# Autodesk Inventor assembly: EPS
(part 2 of 2)
- Mate:673 (12.9 mm): 21-4754:3
- Mate:674 (-12.5 mm): 21-4754:4
- Mate:675 (16.2 mm): 21-4754:4
- Mate:676: 21-1002:1 ↔ EPS_PCB:1
- Mate:677: 21-1002:2 ↔ EPS_PCB:1
- Mate:678: 21-1002:3 ↔ EPS_PCB:1
- Mate:679: 21-1002:4 ↔ EPS_PCB:1
- Mate:680 (-0.3 mm): 21-1002:1
- Mate:681 (63 mm): 21-1002:1
- Mate:682 (-10 mm): 21-1002:2
- Mate:683 (21.2 mm): 21-1002:2
- Mate:684 (16.7 mm): 21-1002:3
- Flush:62 (16.4 mm): 21-1002:3
- Mate:685 (11.3 mm): 21-1002:4
- Mate:686 (89.5 mm): 21-1002:4
- Mate:687: 21-1500:1 ↔ EPS_PCB:1
- Mate:688: 21-1500:2 ↔ EPS_PCB:1
- Mate:689 (-38.6 mm): 21-1500:1
- Mate:690 (46.6 mm): 21-1500:1
- Mate:691 (44.2 mm): 21-1500:2
- Flush:63 (-30.8 mm): 21-1500:2
- Mate:692: 21-1583:1 ↔ EPS_PCB:1
- Mate:693 (-8.9 mm): 21-1583:1
- Mate:694 (84.9 mm): 21-1583:1
- Mate:695: 21-3300:1 ↔ EPS_PCB:1
- Mate:696: 21-3300:2 ↔ EPS_PCB:1
- Mate:697: 21-3603:1 ↔ EPS_PCB:1
- Mate:698: 21-3603:2 ↔ EPS_PCB:1
- Mate:699 (13.5 mm): 21-3300:1
- Flush:64 (-3.1 mm): 21-3300:1
- Mate:700 (9.5 mm): 21-3300:2
- Flush:65 (12.8 mm): 21-3300:2
- Mate:701 (54.1 mm): 21-3603:1
- Flush:66 (-35.9 mm): 21-3603:1
- Mate:702 (-29.7 mm): 21-3603:2
- Mate:703 (58.8 mm): 21-3603:2
- Mate:704: 21-4700:1 ↔ EPS_PCB:1
- Mate:705: 21-4700:2 ↔ EPS_PCB:1
- Mate:706 (37.1 mm): 21-4700:1
- Mate:707 (82.7 mm): 21-4700:1
- Mate:708 (5.2 mm): 21-4700:2
- Flush:67 (43.6 mm): 21-4700:2
- Mate:709: 21-5363:1 ↔ EPS_PCB:1
- Mate:710: 21-6203:1 ↔ EPS_PCB:1
- Mate:711: 21-6203:2 ↔ EPS_PCB:1
- Mate:712: 21-7500:1 ↔ EPS_PCB:1
- Mate:713: 21-7500:2 ↔ EPS_PCB:1
- Mate:714: 21-7500:3 ↔ EPS_PCB:1
- Mate:715: 21-7500:4 ↔ EPS_PCB:1
- Mate:716: 21-7500:5 ↔ EPS_PCB:1
- Mate:717: 21-7500:6 ↔ EPS_PCB:1
- Mate:718 (87.2 mm): 21-5363:1
- Flush:68 (-12.1 mm): 21-5363:1
- Mate:719 (54.1 mm): 21-6203:1
- Flush:69 (-39.3 mm): 21-6203:1
- Mate:720 (55.7 mm): 21-6203:2
- Flush:70 (26.9 mm): 21-6203:2
- Mate:721 (6.7 mm): 21-7500:1
- Mate:722 (21 mm): 21-7500:1
- Mate:723 (4.7 mm): 21-7500:2
- Mate:724 (28.8 mm): 21-7500:2
- Mate:725 (58.5 mm): 21-7500:3
- Flush:71 (-4.2 mm): 21-7500:3
- Mate:726 (57.1 mm): 21-7500:4
- Flush:72 (14.4 mm): 21-7500:4
- Mate:727 (26.7 mm): 21-7500:5
- Mate:728 (21 mm): 21-7500:5
- Mate:729 (21.3 mm): 21-7500:6
- Mate:730 (28.8 mm): 21-7500:6
- Mate:731: 26-0007:1 ↔ EPS_PCB:1
- Mate:732: 26-0007:2 ↔ EPS_PCB:1
- Mate:733: 26-0007:3 ↔ EPS_PCB:1
- Mate:734: 26-0007:4 ↔ EPS_PCB:1
- Mate:735: 26-0007:5 ↔ EPS_PCB:1
- Mate:736: 26-0007:6 ↔ EPS_PCB:1
- Mate:737: 26-0007:7 ↔ EPS_PCB:1
- Mate:738: 26-0007:8 ↔ EPS_PCB:1
- Mate:739: 26-0007:9 ↔ EPS_PCB:1
- Mate:740: 26-0007:10 ↔ EPS_PCB:1
- Mate:741: 26-0007:11 ↔ EPS_PCB:1
- Mate:742: 26-0007:12 ↔ EPS_PCB:1
- Mate:743: 26-0007:13 ↔ EPS_PCB:1
- Mate:744: 26-0007:14 ↔ EPS_PCB:1
- Mate:745: 26-0007:15 ↔ EPS_PCB:1
- Mate:746: 26-0007:16 ↔ EPS_PCB:1
- Mate:747 (39.2 mm): 26-0007:1
- Flush:73 (39.8 mm): 26-0007:1
- Mate:748 (-25.6 mm): 26-0007:2
- Mate:749 (79.9 mm): 26-0007:2
- Mate:750 (-10 mm): 26-0007:3
- Mate:751 (79.6 mm): 26-0007:3
- Mate:752 (28 mm): 26-0007:4
- Flush:74 (43.4 mm): 26-0007:4
- Mate:753 (23.3 mm): 26-0007:5
- Mate:754 (73 mm): 26-0007:5
- Mate:755 (23.3 mm): 26-0007:6
- Mate:756 (70.1 mm): 26-0007:6
- Mate:757 (26.1 mm): 26-0007:7
- Mate:758 (70.1 mm): 26-0007:7
- Mate:759 (26.1 mm): 26-0007:8
- Mate:760 (73 mm): 26-0007:8
- Mate:761 (20.5 mm): 26-0007:9
- Mate:762 (73 mm): 26-0007:9
- Mate:763 (33.2 mm): 26-0007:10
- Flush:75 (34.4 mm): 26-0007:10
- Mate:764 (36.2 mm): 26-0007:11
- Flush:76 (38.1 mm): 26-0007:11
- Mate:765 (30.4 mm): 26-0007:12
- Flush:77 (35.3 mm): 26-0007:12
- Mate:766 (33.2 mm): 26-0007:13
- Flush:78 (37.3 mm): 26-0007:13
- Mate:767 (-7.2 mm): 26-0007:14
- Mate:768 (79.6 mm): 26-0007:14
- Mate:769 (-12.8 mm): 26-0007:15
- Mate:770 (79.6 mm): 26-0007:15
- Mate:771 (-22.8 mm): 26-0007:16
- Mate:772 (79.9 mm): 26-0007:16
- Mate:774: 26-0000:2 ↔ EPS_PCB:1
- Mate:775: 26-0000:3 ↔ EPS_PCB:1
- Mate:776: 26-0000:1 ↔ EPS_PCB:1
- Mate:777 (-9 mm): 26-0000:1
- Flush:79 (-8 mm): 26-0000:1
- Mate:778 (-34.6 mm): 26-0000:2
- Mate:779 (76.9 mm): 26-0000:2
- Mate:780 (-9 mm): 26-0000:3
- Flush:80 (-11.1 mm): 26-0000:3
- Mate:781: 26-0001:1 ↔ EPS_PCB:1
- Mate:782: 26-0001:2 ↔ EPS_PCB:1
- Mate:783 (14.8 mm): 26-0001:1
- Flush:81 (35.2 mm): 26-0001:1
- Mate:784 (56.9 mm): 26-0001:2
- Flush:82 (-23.9 mm): 26-0001:2
- Mate:785: 26-0008:1 ↔ EPS_PCB:1
- Mate:786: 26-0008:2 ↔ EPS_PCB:1
- Mate:787: 26-0008:3 ↔ EPS_PCB:1
- Mate:788: 26-0008:4 ↔ EPS_PCB:1
- Mate:789: 26-0008:5 ↔ EPS_PCB:1
- Mate:790: 26-0008:6 ↔ EPS_PCB:1
- Mate:791: 26-0008:7 ↔ EPS_PCB:1
- Mate:792: 26-0008:8 ↔ EPS_PCB:1
- Mate:793: 26-0008:9 ↔ EPS_PCB:1
- Mate:794: 26-0008:10 ↔ EPS_PCB:1
- Mate:795: 26-0008:11 ↔ EPS_PCB:1
- Mate:796: 26-0008:12 ↔ EPS_PCB:1
- Mate:797 (8.1 mm): 26-0008:1
- Mate:798 (-43.9 mm): 26-0008:1
- Mate:799 (79.9 mm): 26-0008:2
- Mate:800 (-4.9 mm): 26-0008:2
- Mate:801 (16.6 mm): 26-0008:3
- Mate:802 (-4.8 mm): 26-0008:3
- Mate:803 (43.44 mm): 26-0008:4
- Flush:83 (-87.2 mm): 26-0008:4
- Mate:804 (88.6 mm): 26-0008:5
- Mate:805 (-44 mm): 26-0008:5
- Mate:806 (51.3 mm): 26-0008:6
- Mate:807 (27.1 mm): 26-0008:6
- Mate:808 (53.6 mm): 26-0008:7
- Mate:809 (-34.4 mm): 26-0008:7
- Mate:810 (-10.5 mm): 26-0008:8
- Flush:84 (-43.1 mm): 26-0008:8
- Mate:811 (29.4 mm): 26-0008:9
- Mate:812 (19 mm): 26-0008:9
- Mate:813 (21.3 mm): 26-0008:10
- Mate:814 (43.9 mm): 26-0008:10
- Mate:815 (62.3 mm): 26-0008:11
- Mate:816 (-32 mm): 26-0008:11
- Mate:817 (66.4 mm): 26-0008:12
- Mate:818 (40.6 mm): 26-0008:12
- Mate:819: 26-0008:13 ↔ EPS_PCB:1
- Mate:820: 26-0008:14 ↔ EPS_PCB:1
- Mate:821 (35.5 mm): 26-0008:13
- Flush:85 (14.8 mm): 26-0008:13
- Mate:822 (58.5 mm): 26-0008:14
- Flush:86 (-27.2 mm): 26-0008:14
- Mate:823: 11-105A:1 ↔ EPS_PCB:1
- Mate:824: 11-105A:2 ↔ EPS_PCB:1
- Mate:825: 11-105A:3 ↔ EPS_PCB:1
- Mate:826: 11-105A:4 ↔ EPS_PCB:1
- Mate:827: 11-105A:5 ↔ EPS_PCB:1
- Mate:828: 11-105A:6 ↔ EPS_PCB:1
- Mate:829: 11-105A:7 ↔ EPS_PCB:1
- Mate:830: 11-105A:8 ↔ EPS_PCB:1
- Mate:831: 11-105A:9 ↔ EPS_PCB:1
- Mate:832: 11-105A:10 ↔ EPS_PCB:1
- Mate:833: 11-105A:11 ↔ EPS_PCB:1
- Mate:834: 11-105A:12 ↔ EPS_PCB:1
- Mate:835: 11-105A:13 ↔ EPS_PCB:1
- Mate:836: 11-105A:14 ↔ EPS_PCB:1
- Mate:837: 11-105A:15 ↔ EPS_PCB:1
- Mate:838: 11-105A:16 ↔ EPS_PCB:1
- Mate:839: 11-105A:17 ↔ EPS_PCB:1
- Mate:840: 11-105A:18 ↔ EPS_PCB:1
- Mate:841: 11-105A:19 ↔ EPS_PCB:1
- Mate:842: 11-105A:20 ↔ EPS_PCB:1
- Mate:843: 11-105A:21 ↔ EPS_PCB:1
- Mate:844: 11-105A:22 ↔ EPS_PCB:1
- Mate:845: 11-105A:23 ↔ EPS_PCB:1
- Mate:846: 11-105A:24 ↔ EPS_PCB:1
- Mate:847: 11-105A:25 ↔ EPS_PCB:1
- Mate:848: 11-105A:26 ↔ EPS_PCB:1
- Mate:849 (37.6 mm): 11-105A:1
- Mate:850 (32.9 mm): 11-105A:1
- Mate:851 (40.9 mm): 11-105A:2
- Mate:852 (18.8 mm): 11-105A:2
- Mate:853 (-5.5 mm): 11-105A:3
- Flush:87 (-25.8 mm): 11-105A:3
- Mate:854 (-43.3 mm): 11-105A:4
- Flush:88 (-20.2 mm): 11-105A:4
- Mate:855 (23.7 mm): 11-105A:5
- Mate:856 (-38.1 mm): 11-105A:5
- Mate:857 (62.1 mm): 11-105A:6
- Mate:858 (24.9 mm): 11-105A:6
- Mate:859 (14.5 mm): 11-105A:7
- Flush:89 (-53.6 mm): 11-105A:7
- Mate:860 (35.3 mm): 11-105A:8
- Flush:90 (-56.4 mm): 11-105A:8
- Mate:861 (38.2 mm): 11-105A:9
- Flush:91 (-56.4 mm): 11-105A:9
- Mate:862 (34.3 mm): 11-105A:10
- Flush:92 (-73.9 mm): 11-105A:10
- Mate:863 (37.2 mm): 11-105A:11
- Flush:93 (-73.9 mm): 11-105A:11
- Mate:864 (-38.9 mm): 11-105A:12
- Flush:94 (-75.9 mm): 11-105A:12
- Mate:865 (-42.4 mm): 11-105A:13
- Flush:95 (-74.7 mm): 11-105A:13
- Mate:866 (-36.9 mm): 11-105A:14
- Flush:96 (-57.1 mm): 11-105A:14
- Mate:867 (57.7 mm): 11-105A:15
- Mate:868 (-39.2 mm): 11-105A:15
- Mate:869 (63.4 mm): 11-105A:16
- Mate:870 (40.6 mm): 11-105A:16
- Mate:871 (29.9 mm): 11-105A:17
- Flush:97 (-62.8 mm): 11-105A:17
- Mate:872 (65.5 mm): 11-105A:18
- Mate:873 (-32 mm): 11-105A:18
- Mate:874 (-38.4 mm): 11-105A:19
- Flush:98 (-64.7 mm): 11-105A:19
- Mate:875 (33.2 mm): 11-105A:20
- Flush:99 (-67.5 mm): 11-105A:20
- Mate:876 (36.9 mm): 11-105A:21
- Flush:100 (-67.5 mm): 11-105A:21
- Mate:877 (-4.3 mm): 11-105A:22
- Flush:101 (-69.4 mm): 11-105A:22
- Mate:878 (-42.7 mm): 11-105A:23
- Flush:102 (-68.3 mm): 11-105A:23
- Mate:879 (69 mm): 11-105A:24
- Mate:880 (-32 mm): 11-105A:24
- Mate:881 (-4.3 mm): 11-105A:25
- Flush:103 (-63 mm): 11-105A:25
- Mate:882 (67 mm): 11-105A:26
- Mate:883 (2.8 mm): 11-105A:26
- Mate:884: 16-475A:1 ↔ EPS_PCB:1
- Flush:886 (-53.6 mm): 16-475A:1
- Mate:885 (11.1 mm): 16-475A:1
- Mate:886: 11-4.7A:1 ↔ EPS_PCB:1
- Mate:887: 11-4.7A:2 ↔ EPS_PCB:1
- Mate:888: 11-8.0A:1 ↔ EPS_PCB:1
- Mate:889: 11-8.0A:2 ↔ EPS_PCB:1
- Mate:890 (38.7 mm): 11-4.7A:1
- Flush:887 (-51.8 mm): 11-4.7A:1
- Mate:891 (-25.8 mm): 11-4.7A:2
- Flush:888 (-53.4 mm): 11-4.7A:2
- Mate:892 (56.4 mm): 11-8.0A:1
- Mate:893 (-3.1 mm): 11-8.0A:1
- Mate:894 (56.4 mm): 11-8.0A:2
- Mate:895 (-1.4 mm): 11-8.0A:2
- Mate:896: 11-106A:1 ↔ EPS_PCB:1
- Mate:897: 11-106A:2 ↔ EPS_PCB:1
- Mate:898: 11-106A:3 ↔ EPS_PCB:1
- Mate:899: 11-106A:4 ↔ EPS_PCB:1
- Mate:900: 11-106A:5 ↔ EPS_PCB:1
- Mate:901: 11-106A:6 ↔ EPS_PCB:1
- Mate:902: 11-106A:7 ↔ EPS_PCB:1
- Mate:903: 11-106A:8 ↔ EPS_PCB:1
- Mate:904: 11-106A:9 ↔ EPS_PCB:1
- Mate:905: 11-106A:10 ↔ EPS_PCB:1
- Mate:906: 11-106A:11 ↔ EPS_PCB:1
- Mate:907: 11-106A:12 ↔ EPS_PCB:1
- Mate:908: 11-106A:13 ↔ EPS_PCB:1
- Mate:909: 11-106A:14 ↔ EPS_PCB:1
- Mate:910: 11-106A:15 ↔ EPS_PCB:1
- Mate:911: 11-106A:16 ↔ EPS_PCB:1
- Mate:912: 11-106A:17 ↔ EPS_PCB:1
- Mate:913: 11-106A:18 ↔ EPS_PCB:1
- Mate:914: 11-106A:19 ↔ EPS_PCB:1
- Mate:915: 11-106A:20 ↔ EPS_PCB:1
- Mate:916: 11-106A:21 ↔ EPS_PCB:1
- Mate:917: 11-106A:22 ↔ EPS_PCB:1
- Mate:918: 11-106A:23 ↔ EPS_PCB:1
- Mate:919: 11-106A:24 ↔ EPS_PCB:1
- Mate:920: 11-106A:25 ↔ EPS_PCB:1
- Mate:921: 11-106A:26 ↔ EPS_PCB:1
- Mate:922: 11-106A:27 ↔ EPS_PCB:1
- Mate:923: 11-106A:28 ↔ EPS_PCB:1
- Mate:924: 11-106A:29 ↔ EPS_PCB:1
- Mate:925 (4 mm): 11-106A:1
- Flush:889 (-22.8 mm): 11-106A:1
- Mate:926 (9.8 mm): 11-106A:2
- Flush:890 (-22.8 mm): 11-106A:2
- Mate:927 (12.7 mm): 11-106A:3
- Flush:891 (-22.8 mm): 11-106A:3
- Mate:928 (19.6 mm): 11-106A:4
- Flush:892 (-22.8 mm): 11-106A:4
- Mate:929 (16.7 mm): 11-106A:5
- Flush:893 (-22.8 mm): 11-106A:5
- Mate:930 (6.7 mm): 11-106A:6
- Flush:894 (-15 mm): 11-106A:6
- Mate:931 (10.7 mm): 11-106A:7
- Flush:895 (-15 mm): 11-106A:7
- Mate:932 (14.7 mm): 11-106A:8
- Flush:896 (-15 mm): 11-106A:8
- Mate:933 (18.7 mm): 11-106A:9
- Flush:897 (-15 mm): 11-106A:9
- Mate:934 (22.7 mm): 11-106A:10
- Flush:898 (-15 mm): 11-106A:10
- Mate:935 (42.7 mm): 11-106A:11
- Flush:899 (-13 mm): 11-106A:11
- Mate:936 (38.7 mm): 11-106A:12
- Flush:900 (-13 mm): 11-106A:12
- Mate:937 (34.7 mm): 11-106A:13
- Flush:901 (-13 mm): 11-106A:13
- Mate:938 (26.7 mm): 11-106A:14
- Flush:902 (-15 mm): 11-106A:14
- Mate:939 (30.7 mm): 11-106A:15
- Flush:903 (-13 mm): 11-106A:15
- Mate:940 (40.7 mm): 11-106A:16
- Flush:904 (-20.8 mm): 11-106A:16
- Mate:941 (36.7 mm): 11-106A:17
- Flush:905 (-20.8 mm): 11-106A:17
- Mate:942 (32.7 mm): 11-106A:18
- Flush:906 (-20.8 mm): 11-106A:18
- Mate:943 (28.7 mm): 11-106A:19
- Flush:907 (-22.8 mm): 11-106A:19
- Mate:944 (25.4 mm): 11-106A:20
- Flush:908 (-22.8 mm): 11-106A:20
- Mate:945 (84.6 mm): 11-106A:21
- Mate:946 (22.8 mm): 11-106A:21
- Mate:947 (-18.7 mm): 11-106A:22
- Flush:909 (-85.5 mm): 11-106A:22
- Mate:948 (37.6 mm): 11-106A:23
- Mate:949 (37.5 mm): 11-106A:23
- Mate:950 (40.9 mm): 11-106A:24
- Mate:951 (23.4 mm): 11-106A:24
- Mate:952 (-5.5 mm): 11-106A:25
- Flush:910 (-30.4 mm): 11-106A:25
- Mate:953 (20.8 mm): 11-106A:26
- Mate:954 (-38.1 mm): 11-106A:26
- Mate:955 (14.5 mm): 11-106A:27
- Flush:911 (-58.2 mm): 11-106A:27
- Mate:956 (-42.7 mm): 11-106A:28
- Flush:912 (-37.4 mm): 11-106A:28
- Mate:957 (46.3 mm): 11-106A:29
- Mate:958 (-13.8 mm): 11-106A:29
- Mate:959: 11-103A:1 ↔ EPS_PCB:1
- Mate:960: 11-150A:1 ↔ EPS_PCB:1
- Mate:961: 11-150A:2 ↔ EPS_PCB:1
- Mate:962 (56.4 mm): 11-103A:1
- Mate:963 (-4.8 mm): 11-103A:1
- Mate:964 (55.2 mm): 11-150A:1
- Mate:965 (3.8 mm): 11-150A:1
- Mate:966 (55.2 mm): 11-150A:2
- Mate:967 (2 mm): 11-150A:2
- Mate:968: 11-104A:1 ↔ EPS_PCB:1
- Mate:969: 11-104A:2 ↔ EPS_PCB:1
- Mate:970: 11-104A:3 ↔ EPS_PCB:1
- Mate:971: 11-104A:4 ↔ EPS_PCB:1
- Mate:972: 11-104A:5 ↔ EPS_PCB:1
- Mate:973: 11-104A:6 ↔ EPS_PCB:1
- Mate:974: 11-104A:7 ↔ EPS_PCB:1
- Mate:975: 11-104A:8 ↔ EPS_PCB:1
- Mate:976: 11-104A:9 ↔ EPS_PCB:1
- Mate:977: 11-104A:10 ↔ EPS_PCB:1
- Mate:978: 11-104A:11 ↔ EPS_PCB:1
- Mate:979: 11-104A:12 ↔ EPS_PCB:1
- Mate:980: 11-104A:13 ↔ EPS_PCB:1
- Mate:981: 11-104A:14 ↔ EPS_PCB:1
- Mate:982: 11-104A:15 ↔ EPS_PCB:1
- Mate:983: 11-104A:16 ↔ EPS_PCB:1
- Mate:984: 11-104A:17 ↔ EPS_PCB:1
- Mate:985: 11-104A:18 ↔ EPS_PCB:1
- Mate:986: 11-104A:19 ↔ EPS_PCB:1
- Mate:987: 11-104A:20 ↔ EPS_PCB:1
- Mate:988: 11-104A:21 ↔ EPS_PCB:1
- Mate:989: 11-104A:22 ↔ EPS_PCB:1
- Mate:990: 11-104A:23 ↔ EPS_PCB:1
- Mate:991: 11-104A:24 ↔ EPS_PCB:1
- Mate:992: 11-104A:25 ↔ EPS_PCB:1
- Mate:993: 11-104A:26 ↔ EPS_PCB:1
- Mate:994: 11-104A:27 ↔ EPS_PCB:1
- Mate:995: 11-104A:28 ↔ EPS_PCB:1
- Mate:996: 11-104A:29 ↔ EPS_PCB:1
- Mate:997: 11-104A:30 ↔ EPS_PCB:1
- Mate:998: 11-104A:31 ↔ EPS_PCB:1
- Mate:999: 11-104A:32 ↔ EPS_PCB:1
- Mate:1000: 11-104A:33 ↔ EPS_PCB:1
- Mate:1001: 11-104A:34 ↔ EPS_PCB:1
- Mate:1002: 11-104A:35 ↔ EPS_PCB:1
- Mate:1003: 11-104A:36 ↔ EPS_PCB:1
- Mate:1004: 11-104A:37 ↔ EPS_PCB:1
- Mate:1005: 11-104A:38 ↔ EPS_PCB:1
- Mate:1006: 11-104A:39 ↔ EPS_PCB:1
- Mate:1007: 11-104A:40 ↔ EPS_PCB:1
- Mate:1008: 11-104A:41 ↔ EPS_PCB:1
- Mate:1009: 11-104A:42 ↔ EPS_PCB:1
- Mate:1010: 11-104A:43 ↔ EPS_PCB:1
- Mate:1011: 11-104A:44 ↔ EPS_PCB:1
- Mate:1012: 11-104A:45 ↔ EPS_PCB:1
- Mate:1013: 11-104A:46 ↔ EPS_PCB:1
- Mate:1014: 11-104A:47 ↔ EPS_PCB:1
- Mate:1015: 11-104A:48 ↔ EPS_PCB:1
- Mate:1016: 11-104A:49 ↔ EPS_PCB:1
- Mate:1017: 11-104A:50 ↔ EPS_PCB:1
- Mate:1018: 11-104A:51 ↔ EPS_PCB:1
- Mate:1019: 11-104A:52 ↔ EPS_PCB:1
- Mate:1020: 11-104A:53 ↔ EPS_PCB:1
- Mate:1021: 11-104A:54 ↔ EPS_PCB:1
- Mate:1022: 11-104A:55 ↔ EPS_PCB:1
- Mate:1023: 11-104A:56 ↔ EPS_PCB:1
- Mate:1024: 11-104A:57 ↔ EPS_PCB:1
- Mate:1025: 11-104A:58 ↔ EPS_PCB:1
- Mate:1026: 11-104A:59 ↔ EPS_PCB:1
- Mate:1027: 11-104A:60 ↔ EPS_PCB:1
- Mate:1028: 11-104A:61 ↔ EPS_PCB:1
- Mate:1029: 11-104A:62 ↔ EPS_PCB:1
- Mate:1030: 11-104A:63 ↔ EPS_PCB:1
- Mate:1031 (5.3 mm): 11-104A:1
- Flush:913 (-65.1 mm): 11-104A:1
- Mate:1032 (58.5 mm): 11-104A:2
- Mate:1033 (5.9 mm): 11-104A:2
- Mate:1034 (39.5 mm): 11-104A:3
- Mate:1035 (26.3 mm): 11-104A:3
- Mate:1036 (39.4 mm): 11-104A:4
- Flush:914 (-76.7 mm): 11-104A:4
- Mate:1037 (-39.9 mm): 11-104A:5
- Flush:915 (-7.7 mm): 11-104A:5
- Mate:1038 (35.1 mm): 11-104A:6
- Flush:916 (-76.7 mm): 11-104A:6
- Mate:1039 (3.5 mm): 11-104A:7
- Mate:1040 (-37.6 mm): 11-104A:7
- Mate:1041 (-36.2 mm): 11-104A:8
- Flush:917 (-89.2 mm): 11-104A:8
- Mate:1042 (85.8 mm): 11-104A:9
- Mate:1043 (-33.8 mm): 11-104A:9
- Mate:1044 (36.3 mm): 11-104A:10
- Mate:1045 (-40.4 mm): 11-104A:10
- Mate:1046 (10.6 mm): 11-104A:11
- Mate:1047 (3.1 mm): 11-104A:11
- Mate:1048 (84.6 mm): 11-104A:12
- Mate:1049 (18.2 mm): 11-104A:12
- Mate:1050 (84.4 mm): 11-104A:13
- Mate:1051 (-21 mm): 11-104A:13
- Mate:1052 (20.5 mm): 11-104A:14
- Flush:918 (-84 mm): 11-104A:14
- Mate:1053 (79 mm): 11-104A:15
- Mate:1054 (-15.1 mm): 11-104A:15
- Mate:1055 (-18.7 mm): 11-104A:16
- Flush:919 (-83.8 mm): 11-104A:16
- Mate:1056 (34 mm): 11-104A:17
- Flush:920 (-29.8 mm): 11-104A:17
- Mate:1057 (35.2 mm): 11-104A:18
- Flush:921 (-37 mm): 11-104A:18
- Mate:1058 (35.5 mm): 11-104A:19
- Mate:1059 (17.5 mm): 11-104A:19
- Mate:1060 (21.1 mm): 11-104A:20
- Flush:922 (-40.3 mm): 11-104A:20
- Mate:1061 (-0.1 mm): 11-104A:21
- Flush:923 (-24.5 mm): 11-104A:21
- Mate:1062 (28.1 mm): 11-104A:22
- Mate:1063 (-4.9 mm): 11-104A:22
- Mate:1064 (19.6 mm): 11-104A:23
- Flush:924 (-52.3 mm): 11-104A:23
- Mate:1065 (55.9 mm): 11-104A:24
- Mate:1066 (15.1 mm): 11-104A:24
- Mate:1067 (15.4 mm): 11-104A:25
- Mate:1068 (-44 mm): 11-104A:25
- Mate:1069 (-40.4 mm): 11-104A:26
- Flush:925 (-20.2 mm): 11-104A:26
- Mate:1070 (17.9 mm): 11-104A:27
- Flush:926 (-60.1 mm): 11-104A:27
- Mate:1071 (23.7 mm): 11-104A:28
- Mate:1072 (-43.9 mm): 11-104A:28
- Mate:1073 (87.8 mm): 11-104A:29
- Mate:1074 (-22.6 mm): 11-104A:29
- Mate:1075 (87.8 mm): 11-104A:30
- Mate:1076 (-20.9 mm): 11-104A:30
- Mate:1077 (-10.5 mm): 11-104A:31
- Flush:927 (-7.6 mm): 11-104A:31
- Mate:1078 (-7.6 mm): 11-104A:32
- Flush:928 (-7.6 mm): 11-104A:32
- Mate:1079 (-34.6 mm): 11-104A:33
- Flush:929 (-79.2 mm): 11-104A:33
- Mate:1080 (83 mm): 11-104A:34
- Mate:1081 (-28.3 mm): 11-104A:34
- Mate:1082 (83.5 mm): 11-104A:35
- Mate:1083 (-6.6 mm): 11-104A:35
- Mate:1084 (47.3 mm): 11-104A:36
- Mate:1085 (5.4 mm): 11-104A:36
- Mate:1086 (46.8 mm): 11-104A:37
- Mate:1087 (-9.9 mm): 11-104A:37
- Mate:1088 (39.7 mm): 11-104A:38
- Mate:1089 (-9.9 mm): 11-104A:38
- Mate:1090 (1.2 mm): 11-104A:39
- Flush:930 (-36.1 mm): 11-104A:39
- Mate:1091 (76.9 mm): 11-104A:40
- Mate:1092 (8.8 mm): 11-104A:40
- Mate:1093 (87 mm): 11-104A:41
- Mate:1094 (24.9 mm): 11-104A:41
- Mate:1095 (54.8 mm): 11-104A:42
- Mate:1096 (8.3 mm): 11-104A:42
- Mate:1097 (-25.7 mm): 11-104A:43
- Flush:931 (-36.6 mm): 11-104A:43
- Mate:1098 (61.2 mm): 11-104A:44
- Mate:1099 (-42.2 mm): 11-104A:44
- Mate:1100 (79 mm): 11-104A:45
- Mate:1101 (24.1 mm): 11-104A:45
- Mate:1102 (-42.7 mm): 11-104A:46
- Flush:932 (-35.7 mm): 11-104A:46
- Mate:1103 (-39.8 mm): 11-104A:47
- Flush:933 (-28.5 mm): 11-104A:47
- Mate:1104 (-12.1 mm): 11-104A:48
- Flush:934 (-11.8 mm): 11-104A:48
- Mate:1105 (-16.22 mm): 11-104A:49
- Flush:935 (-47.2 mm): 11-104A:49
- Mate:1106 (40.8 mm): 11-104A:50
- Mate:1107 (-15.2 mm): 11-104A:50
- Mate:1108 (43.4 mm): 11-104A:51
- Flush:936 (-10.9 mm): 11-104A:51
- Mate:1109 (22.5 mm): 11-104A:52
- Flush:937 (-22.8 mm): 11-104A:52
- Mate:1110 (-15.8 mm): 11-104A:53
- Flush:938 (-21.5 mm): 11-104A:53
- Mate:1111 (-12.9 mm): 11-104A:54
- Flush:939 (-21.5 mm): 11-104A:54
- Mate:1112 (61.2 mm): 11-104A:55
- Mate:1113 (42.3 mm): 11-104A:55
- Mate:1114 (6.9 mm): 11-104A:56
- Flush:940 (-22.8 mm): 11-104A:56
- Mate:1115 (29.4 mm): 11-104A:57
- Mate:1116 (14.4 mm): 11-104A:57
- Mate:1117 (73 mm): 11-104A:58
- Mate:1118 (12 mm): 11-104A:58
- Mate:1119 (-43.3 mm): 11-104A:59
- Flush:941 (-41.6 mm): 11-104A:59
- Mate:1120 (36.1 mm): 11-104A:60
- Mate:1121 (-35.8 mm): 11-104A:60
- Mate:1122 (17.6 mm): 11-104A:61
- Flush:942 (-73.6 mm): 11-104A:61
- Mate:1123 (-10.8 mm): 11-104A:62
- Flush:943 (-60 mm): 11-104A:62
- Mate:1124 (-10.8 mm): 11-104A:63
- Flush:944 (-54.2 mm): 11-104A:63
- Mate:1125: 11-471A:1 ↔ EPS_PCB:1
- Mate:1126: 11-471A:2 ↔ EPS_PCB:1
- Mate:1127 (-41.7 mm): 11-471A:1
- Flush:945 (-46.6 mm): 11-471A:1
- Mate:1128 (41.3 mm): 11-471A:2
- Mate:1129 (30.8 mm): 11-471A:2
- Mate:1130: 34-472A:1 ↔ EPS_PCB:1
- Mate:1131: 34-472A:2 ↔ EPS_PCB:1
- Mate:1132 (35.9 mm): 34-472A:1
- Mate:1133 (46.7 mm): 34-472A:1
- Mate:1134 (-32.9 mm): 34-472A:2
- Mate:1135 (47.9 mm): 34-472A:2
- Mate:1136: 40-805A:1 ↔ EPS_PCB:1
- Mate:1137 (-2.4 mm): 40-805A:1
- Flush:946 (-52.7 mm): 40-805A:1
- Mate:1138: 23-0.01:1 ↔ EPS_PCB:1
- Mate:1139: 23-0.01:2 ↔ EPS_PCB:1
- Mate:1140 (49.8 mm): 23-0.01:1
- Mate:1141 (-38.4 mm): 23-0.01:1
- Mate:1142 (43.3 mm): 23-0.01:2
- Mate:1143 (28.7 mm): 23-0.01:2
- Mate:1144: 23-0.01:4 ↔ EPS_PCB:1
- Mate:1145: 23-0.01:3 ↔ EPS_PCB:1
- Mate:1146 (13.3 mm): 23-0.01:3
- Mate:1147 (14.3 mm): 23-0.01:3
- Mate:1148 (15.3 mm): 23-0.01:4
- Flush:947 (14.3 mm): 23-0.01:4
- Mate:1149: 23-12m0:8 ↔ EPS_PCB:1
- Mate:1150: 23-12m0:7 ↔ EPS_PCB:1
- Mate:1151: 23-12m0:6 ↔ EPS_PCB:1
- Mate:1152: 23-12m0:5 ↔ EPS_PCB:1
- Mate:1153: 23-12m0:4 ↔ EPS_PCB:1
- Mate:1154: 23-12m0:3 ↔ EPS_PCB:1
- Mate:1155: 23-12m0:2 ↔ EPS_PCB:1
- Mate:1156: 23-12m0:1 ↔ EPS_PCB:1
- Mate:1157 (49.8 mm): 23-12m0:5
- Flush:948 (41 mm): 23-12m0:5
- Mate:1158 (40 mm): 23-12m0:6
- Flush:949 (-43.1 mm): 23-12m0:6
- Mate:1159 (43.3 mm): 23-12m0:7
- Flush:950 (-26 mm): 23-12m0:7
- Mate:1160 (-25.5 mm): 23-12m0:8
- Mate:1161 (42.4 mm): 23-12m0:8
- Mate:1162 (86.8 mm): 23-12m0:1
- Mate:1163 (-27.7 mm): 23-12m0:1
- Mate:1164 (86.8 mm): 23-12m0:2
- Mate:1165 (-14.3 mm): 23-12m0:2
- Mate:1166 (84.8 mm): 23-12m0:3
- Mate:1167 (14.3 mm): 23-12m0:3
- Mate:1168 (84.8 mm): 23-12m0:4
- Mate:1169 (27.7 mm): 23-12m0:4
- Mate:1170: 40-323A:1 ↔ EPS_PCB:1
- Mate:1171 (2.9 mm): 40-323A:1
- Flush:951 (-52.4 mm): 40-323A:1
- Mate:1172: 16-227A:1 ↔ EPS_PCB:1
- Mate:1173: 16-227A:2 ↔ EPS_PCB:1
- Mate:1174: 16-227A:3 ↔ EPS_PCB:1
- Flush:952 (-47 mm): 16-227A:1
- Mate:1175 (42.3 mm): 16-227A:1
- Flush:953 (-48.3 mm): 16-227A:2
- Mate:1176 (-26.5 mm): 16-227A:2
- Mate:1177 (-12.5 mm): 16-227A:3
- Mate:1178 (87.9 mm): 16-227A:3
- Mate:1179: 27-0003:1 ↔ EPS_PCB:1
- Mate:1180: 27-0003:2 ↔ EPS_PCB:1
- Mate:1181: 27-0003:3 ↔ EPS_PCB:1
- Mate:1182: 27-0003:4 ↔ EPS_PCB:1
- Mate:1183: 27-0003:5 ↔ EPS_PCB:1
- Flush:954 (-33.4 mm): 27-0003:1
- Mate:1184 (35.2 mm): 27-0003:1
- Mate:1185 (-40.4 mm): 27-0003:2
- Flush:955 (-16.6 mm): 27-0003:2
- Mate:1186 (21.1 mm): 27-0003:3
- Flush:956 (-36.7 mm): 27-0003:3
- Mate:1187 (28.1 mm): 27-0003:4
- Mate:1188 (-1.3 mm): 27-0003:4
- Mate:1189 (55.9 mm): 27-0003:5
- Mate:1190 (18.7 mm): 27-0003:5
- Mate:1191: 27-0004:1 ↔ EPS_PCB:1
- Mate:1192: 27-0004:2 ↔ EPS_PCB:1
- Mate:1193: 27-0004:3 ↔ EPS_PCB:1
- Mate:1194 (80.2 mm): 27-0004:1
- Mate:1195 (20.3 mm): 27-0004:1
- Mate:1196 (80.2 mm): 27-0004:2
- Mate:1197 (-18.7 mm): 27-0004:2
- Mate:1198 (32.1 mm): 27-0004:3
- Mate:1199 (-41.5 mm): 27-0004:3
- Mate:1200: 08-0002:1 ↔ EPS_PCB:1
- Mate:1201: 08-0002:2 ↔ EPS_PCB:1
- Mate:1202: 08-0002:3 ↔ EPS_PCB:1
- Mate:1203 (-41 mm): 08-0002:1
- Flush:957 (-24.3 mm): 08-0002:1
- Flush:958 (12.4 mm): 08-0002:2
- Mate:1204 (83.4 mm): 08-0002:2
- Mate:1205 (62.6 mm): 08-0002:3
- Mate:1206 (21.7 mm): 08-0002:3
- Mate:1207: 60-0006:1 ↔ EPS_PCB:1
- Mate:1208: 60-0006:2 ↔ EPS_PCB:1
- Mate:1209 (14 mm): 60-0006:1
- Mate:1210 (-12.2 mm): 60-0006:1
- Mate:1211 (5.6 mm): 60-0006:2
- Flush:959 (-10.7 mm): 60-0006:2
- Mate:1212: 56-0002:1 ↔ EPS_PCB:1
- Mate:1213: 56-0002:2 ↔ EPS_PCB:1
- Mate:1214: 56-0002:3 ↔ EPS_PCB:1
- Mate:1215: 56-0002:4 ↔ EPS_PCB:1
- Flush:960 (-80.2 mm): 56-0002:1
- Mate:1216 (28.4 mm): 56-0002:1
- Flush:961 (-82.2 mm): 56-0002:2
- Mate:1217 (-28.4 mm): 56-0002:2
- Mate:1218 (-37.5 mm): 56-0002:3
- Flush:962 (-54.2 mm): 56-0002:3
- Mate:1219 (29.4 mm): 56-0002:4
- Flush:963 (-47.7 mm): 56-0002:4
- Mate:1220: 56-0007:1 ↔ EPS_PCB:1
- Mate:1221: 56-0007:2 ↔ EPS_PCB:1
- Mate:1222 (14.4 mm): 56-0007:1
- Flush:964 (-87.3 mm): 56-0007:1
- Mate:1223 (-10 mm): 56-0007:2
- Flush:965 (-18.7 mm): 56-0007:2
- Mate:1224: 56-0005:2 ↔ EPS_PCB:1
- Mate:1225: 56-0005:1 ↔ EPS_PCB:1
- Mate:1226 (11 mm): 56-0005:1
- Flush:966 (-11.6 mm): 56-0005:1
- Mate:1227 (-11 mm): 56-0005:2
- Mate:1228 (14.1 mm): 56-0005:2
- Flush:967 (-84.35 mm): 49-0004:1
- Mate:1229 (8.845 mm): 49-0004:1
- Mate:1230: 63-0001:1 ↔ EPS_PCB:1
- Mate:1231: 63-0001:2 ↔ EPS_PCB:1
- Mate:1232: 63-0001:3 ↔ EPS_PCB:1
- Mate:1233: 63-0001:4 ↔ EPS_PCB:1
- Mate:1234: 63-0001:5 ↔ EPS_PCB:1
- Mate:1235 (81.4 mm): 63-0001:1
- Mate:1236 (-31.3 mm): 63-0001:1
- Mate:1237 (31.6 mm): 63-0001:2
- Mate:1238 (39.4 mm): 63-0001:2
- Mate:1239 (6.3 mm): 63-0001:3
- Mate:1240 (42.6 mm): 63-0001:3
- Mate:1241 (38.6 mm): 63-0001:4
- Mate:1242 (-34.6 mm): 63-0001:4
- Mate:1243 (79.4 mm): 63-0001:5
- Mate:1244 (31.3 mm): 63-0001:5
- Mate:1245: 08-0003:8 ↔ EPS_PCB:1
- Mate:1246: 08-0003:7 ↔ EPS_PCB:1
- Mate:1247: 08-0003:6 ↔ EPS_PCB:1
- Mate:1248: 08-0003:5 ↔ EPS_PCB:1
- Mate:1249: 08-0003:4 ↔ EPS_PCB:1
- Mate:1250: 08-0003:3 ↔ EPS_PCB:1
- Mate:1251: 08-0003:2 ↔ EPS_PCB:1
- Mate:1252: 08-0003:1 ↔ EPS_PCB:1
- Mate:1253 (87 mm): 08-0003:1
- Mate:1254 (27.4 mm): 08-0003:1
- Flush:968 (-87.8 mm): 08-0003:2
- Flush:969 (25.1 mm): 08-0003:2
- Mate:1255 (73.1 mm): 08-0003:3
- Mate:1256 (14.5 mm): 08-0003:3
- Mate:1257 (17.6 mm): 08-0003:4
- Flush:970 (-71.1 mm): 08-0003:4
- Flush:971 (36.9 mm): 08-0003:5
- Mate:1258 (39.2 mm): 08-0003:5
- Flush:972 (43.5 mm): 08-0003:6
- Mate:1259 (44.1 mm): 08-0003:6
- Mate:1260 (87.8 mm): 08-0003:7
- Mate:1261 (-18.4 mm): 08-0003:7
- Mate:1262 (83 mm): 08-0003:8
- Mate:1263 (-25.8 mm): 08-0003:8
- Mate:1264: 60-0015:1 ↔ EPS_PCB:1
- Mate:1265: 60-0015:2 ↔ EPS_PCB:1
- Mate:1266: 60-0015:3 ↔ EPS_PCB:1
- Mate:1267: 60-0015:4 ↔ EPS_PCB:1
- Mate:1268: 60-0015:5 ↔ EPS_PCB:1
- Mate:1269: 60-0015:6 ↔ EPS_PCB:1
- Mate:1270: 60-0015:7 ↔ EPS_PCB:1
- Mate:1271: 60-0015:8 ↔ EPS_PCB:1
- Mate:1272: 60-0015:9 ↔ EPS_PCB:1
- Mate:1273: 60-0015:10 ↔ EPS_PCB:1
- Mate:1274: 60-0015:11 ↔ EPS_PCB:1
- Mate:1275: 60-0015:12 ↔ EPS_PCB:1
- Mate:1276: 60-0015:13 ↔ EPS_PCB:1
- Mate:1277: 60-0015:14 ↔ EPS_PCB:1
- Mate:1278: 60-0015:15 ↔ EPS_PCB:1
- Mate:1279: 60-0015:16 ↔ EPS_PCB:1
- Mate:1280: 60-0015:17 ↔ EPS_PCB:1
- Mate:1281: 60-0015:18 ↔ EPS_PCB:1
- Mate:1282: 60-0015:19 ↔ EPS_PCB:1
- Mate:1283: 60-0015:20 ↔ EPS_PCB:1
- Mate:1284 (30.1 mm): 60-0015:1
- Flush:973 (-59.6 mm): 60-0015:1
- Mate:1285 (38.1 mm): 60-0015:2
- Flush:974 (-59.6 mm): 60-0015:2
- Mate:1286 (33.7 mm): 60-0015:3
- Flush:975 (-64.3 mm): 60-0015:3
- Flush:1288 (-32.7 mm): 60-0015:4
- Mate:1287 (70.7 mm): 60-0015:4
- Flush:1289 (-29.7 mm): 60-0015:5
- Mate:1288 (66 mm): 60-0015:5
- Flush:1290 (-37.7 mm): 60-0015:6
- Mate:1289 (64.3 mm): 60-0015:6
- Flush:1291 (-36.7 mm): 60-0015:7
- Mate:1290 (70.7 mm): 60-0015:7
- Mate:1291 (-38.9 mm): 60-0015:8
- Flush:1292 (-61.5 mm): 60-0015:8
- Mate:1292 (-42.9 mm): 60-0015:9
- Flush:1293 (-65.1 mm): 60-0015:9
- Mate:1293 (-34.9 mm): 60-0015:10
- Flush:1294 (-60.3 mm): 60-0015:10
- Mate:1294 (-34.9 mm): 60-0015:11
- Flush:1295 (-65 mm): 60-0015:11
- Flush:1296 (42.9 mm): 60-0015:12
- Mate:1295 (71.5 mm): 60-0015:12
- Flush:1297 (38.9 mm): 60-0015:13
- Mate:1296 (67.9 mm): 60-0015:13
- Flush:1298 (38.9 mm): 60-0015:14
- Mate:1297 (72.7 mm): 60-0015:14
- Flush:1299 (34.9 mm): 60-0015:15
- Mate:1298 (69.7 mm): 60-0015:15
- Mate:1299 (-0.1 mm): 60-0015:16
- Flush:1300 (-66.2 mm): 60-0015:16
- Mate:1300 (-4.1 mm): 60-0015:17
- Flush:1301 (-66.2 mm): 60-0015:17
- Mate:1301 (83.7 mm): 60-0015:18
- Mate:1302 (13.6 mm): 60-0015:18
- Mate:1303 (79.7 mm): 60-0015:19
- Mate:1304 (13.6 mm): 60-0015:19
- Mate:1305 (34.1 mm): 60-0015:20
- Flush:1302 (-59.6 mm): 60-0015:20
- Mate:1306: 51-0002:1 ↔ EPS_PCB:1
- Mate:1307: 51-0002:2 ↔ EPS_PCB:1
- Flush:1309 (-33.4 mm): 51-0002:1
- Flush:1310 (-40.8 mm): 51-0002:1
- Mate:1308 (44 mm): 51-0002:2
- Flush:1311 (38.8 mm): 51-0002:2
- Mate:1309: 51-0001:1 ↔ EPS_PCB:1
- Mate:1310 (0.3 mm): 51-0001:1
- Mate:1311 (69.9 mm): 51-0001:1
- Mate:1312: 61-0002:1 ↔ EPS_PCB:1
- Flush:1312 (2.3 mm): 61-0002:1
- Flush:1313 (-43.8 mm): 61-0002:1
- Mate:1313: 60-0014:26 ↔ EPS_PCB:1
- Mate:1314: 60-0014:25 ↔ EPS_PCB:1
- Mate:1315: 60-0014:24 ↔ EPS_PCB:1
- Mate:1316: 60-0014:23 ↔ EPS_PCB:1
- Mate:1317: 60-0014:22 ↔ EPS_PCB:1
- Mate:1318: 60-0014:21 ↔ EPS_PCB:1
- Mate:1319: 60-0014:20 ↔ EPS_PCB:1
- Mate:1320: 60-0014:19 ↔ EPS_PCB:1
- Mate:1321: 60-0014:18 ↔ EPS_PCB:1
- Mate:1322: 60-0014:17 ↔ EPS_PCB:1
- Mate:1323: 60-0014:16 ↔ EPS_PCB:1
- Mate:1324: 60-0014:15 ↔ EPS_PCB:1
- Mate:1325: 60-0014:14 ↔ EPS_PCB:1
- Mate:1326: 60-0014:13 ↔ EPS_PCB:1
- Mate:1327: 60-0014:12 ↔ EPS_PCB:1
- Mate:1328: 60-0014:11 ↔ EPS_PCB:1
- Mate:1329: 60-0014:10 ↔ EPS_PCB:1
- Mate:1330: 60-0014:9 ↔ EPS_PCB:1
- Mate:1331: 60-0014:8 ↔ EPS_PCB:1
- Mate:1332: 60-0014:7 ↔ EPS_PCB:1
- Mate:1333: 60-0014:6 ↔ EPS_PCB:1
- Mate:1334: 60-0014:5 ↔ EPS_PCB:1
- Mate:1335: 60-0014:4 ↔ EPS_PCB:1
- Mate:1336: 60-0014:3 ↔ EPS_PCB:1
- Mate:1337: 60-0014:2 ↔ EPS_PCB:1
- Mate:1338: 60-0014:1 ↔ EPS_PCB:1
- Flush:1314 (16.8 mm): 60-0014:1
- Mate:1339 (44.3 mm): 60-0014:1
- Mate:1340 (16 mm): 60-0014:2
- Mate:1341 (42.9 mm): 60-0014:2
- Mate:1342 (23.8 mm): 60-0014:3
- Mate:1343 (40.9 mm): 60-0014:3
- Mate:1344 (16 mm): 60-0014:4
- Mate:1345 (38.9 mm): 60-0014:4
- Mate:1346 (23.8 mm): 60-0014:5
- Mate:1347 (36.9 mm): 60-0014:5
- Mate:1348 (16 mm): 60-0014:6
- Mate:1349 (34.9 mm): 60-0014:6
- Mate:1350 (23.8 mm): 60-0014:7
- Mate:1351 (32.9 mm): 60-0014:7
- Mate:1352 (16 mm): 60-0014:8
- Mate:1353 (30.9 mm): 60-0014:8
- Mate:1354 (25.8 mm): 60-0014:9
- Mate:1355 (28.9 mm): 60-0014:9
- Mate:1356 (18 mm): 60-0014:10
- Mate:1357 (26.9 mm): 60-0014:10
- Mate:1358 (25.8 mm): 60-0014:11
- Mate:1359 (24.9 mm): 60-0014:11
- Mate:1360 (18 mm): 60-0014:12
- Mate:1361 (22.9 mm): 60-0014:12
- Mate:1362 (25.8 mm): 60-0014:13
- Mate:1363 (20.9 mm): 60-0014:13
- Mate:1364 (18 mm): 60-0014:14
- Mate:1365 (18.9 mm): 60-0014:14
- Mate:1366 (25.8 mm): 60-0014:15
- Mate:1367 (16.9 mm): 60-0014:15
- Mate:1368 (18 mm): 60-0014:16
- Mate:1369 (14.9 mm): 60-0014:16
- Mate:1370 (25.8 mm): 60-0014:17
- Mate:1371 (12.9 mm): 60-0014:17
- Mate:1372 (18 mm): 60-0014:18
- Mate:1373 (10.9 mm): 60-0014:18
- Mate:1374 (25.8 mm): 60-0014:19
- Mate:1375 (8.9 mm): 60-0014:19
- Mate:1376 (18 mm): 60-0014:20
- Mate:1377 (6.9 mm): 60-0014:20
- Mate:1378 (25.8 mm): 60-0014:21
- Mate:1379 (4.9 mm): 60-0014:21
- Flush:1315 (-4.6 mm): 60-0014:22
- Mate:1380 (62.2 mm): 60-0014:22
- Flush:1316 (11.4 mm): 60-0014:23
- Mate:1381 (57.1 mm): 60-0014:23
- Mate:1382 (79.7 mm): 60-0014:24
- Mate:1383 (37.1 mm): 60-0014:24
- Flush:1317 (40.6 mm): 60-0014:25
- Mate:1384 (4.8 mm): 60-0014:25
- Flush:1318 (36.8 mm): 60-0014:26
- Mate:1385 (86.3 mm): 60-0014:26
- Mate:1386: 60-0004:1 ↔ EPS_PCB:1
- Mate:1387: 60-0004:2 ↔ EPS_PCB:1
- Mate:1388: 09-0001:1 ↔ EPS_PCB:1
- Mate:1389: 09-0001:2 ↔ EPS_PCB:1
- Mate:1390: 09-0001:3 ↔ EPS_PCB:1
- Mate:1391: 09-0001:4 ↔ EPS_PCB:1
- Mate:1392: 09-0001:5 ↔ EPS_PCB:1
- Flush:1319 (-31.8 mm): 60-0004:1
- Mate:1393 (53.8 mm): 60-0004:1
- Flush:1320 (31.5 mm): 60-0004:2
- Mate:1394 (55.6 mm): 60-0004:2
- Mate:1395 (19.4 mm): 09-0001:1
- Mate:1396 (-15.8 mm): 09-0001:1
- Mate:1397 (19.4 mm): 09-0001:2
- Mate:1398 (-12.9 mm): 09-0001:2
- Flush:1321 (-81.3 mm): 09-0001:3
- Flush:1322 (34.6 mm): 09-0001:3
- Flush:1323 (-9.7 mm): 09-0001:4
- Flush:1324 (10.5 mm): 09-0001:4
- Flush:1325 (-9.7 mm): 09-0001:5
- Flush:1326 (7.6 mm): 09-0001:5
- Mate:1399: 13-106A:1 ↔ EPS_PCB:1
- Mate:1400: 13-106A:2 ↔ EPS_PCB:1
- Mate:1401: 13-106A:3 ↔ EPS_PCB:1
- Mate:1402: 13-106A:4 ↔ EPS_PCB:1
- Mate:1403: 13-106A:5 ↔ EPS_PCB:1
- Mate:1404: 13-106A:6 ↔ EPS_PCB:1
- Mate:1405: 13-106A:7 ↔ EPS_PCB:1
- Mate:1406: 13-106A:8 ↔ EPS_PCB:1
- Mate:1407 (24.8 mm): 13-106A:1
- Flush:1327 (-46.9 mm): 13-106A:1
- Mate:1408 (38.9 mm): 13-106A:2
- Flush:1328 (-41.1 mm): 13-106A:2
- Mate:1409 (37.5 mm): 13-106A:3
- Mate:1410 (39.6 mm): 13-106A:3
- Mate:1411 (21.8 mm): 13-106A:4
- Flush:1329 (-44.4 mm): 13-106A:4
- Mate:1412 (-34.8 mm): 13-106A:5
- Flush:1330 (-42.4 mm): 13-106A:5
- Mate:1413 (-30.2 mm): 13-106A:6
- Flush:1331 (-42.4 mm): 13-106A:6
- Mate:1414 (49.8 mm): 13-106A:7
- Mate:1415 (-43.6 mm): 13-106A:7
- Mate:1416 (-42.1 mm): 13-106A:8
- Flush:1332 (-53.4 mm): 13-106A:8
- Mate:1417: 36-152A:1 ↔ EPS_PCB:1
- Mate:1418 (51.9 mm): 36-152A:1
- Mate:1419 (8.3 mm): 36-152A:1
- Insert:27: EPS_RegulatorHeatsink-A:1 ↔ EPS_PCB:1
- Insert:28: EPS_RegulatorHeatsink-A:1 ↔ EPS_PCB:1
- Insert:29: EPS_RegulatorHeatsink-B:1 ↔ EPS_PCB:1
- Insert:30: EPS_RegulatorHeatsink-B:1 ↔ EPS_PCB:1
